# Autodesk Inventor assembly: ElectronicsHousing
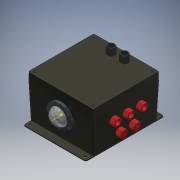
[picture p0: Inventor's stored thumbnail of the model, 180x180]
Saved by Autodesk Inventor 2018 (Build 220112000, 112)
## iProperties
Created: 2019-02-20
Part Number: ElectronicsHousing
Document SubType Name: Assembly
Designer: anirudh
Author: anirudh
## Documents named in this file (10)
- C:\Users\anirudh\Documents\MARS Fund\MATE Robotics\Silicon Sharks\2018-2019\ElectronicsHousing\ElectronicsHousing.iam
- C:\Users\anirudh\Documents\MARS Fund\MATE Robotics\Silicon Sharks\2018-2019\ElectronicsHousing\AluminumHousing(Master).ipt
- C:\Users\anirudh\Documents\MARS Fund\MATE Robotics\Silicon Sharks\2018-2019\ElectronicsHousing\Dome(2in)\2inDome.iam
- C:\Users\anirudh\Documents\MARS Fund\MATE Robotics\Silicon Sharks\2018-2019\ElectronicsHousing\Dome(2in)\DomeGasket.ipt
- C:\Users\anirudh\Documents\MARS Fund\MATE Robotics\Silicon Sharks\2018-2019\ElectronicsHousing\PENETRATOR-M-BOLT-6MM-10-25-R2.ipt
- C:\Users\anirudh\Documents\MARS Fund\MATE Robotics\Silicon Sharks\2018-2019\ElectronicsHousing\6mmPenetratorORing.ipt
- C:\Users\anirudh\Documents\MARS Fund\MATE Robotics\Silicon Sharks\2018-2019\ElectronicsHousing\PENETRATOR-M-BOLT-8MM-10-25-R1.ipt
- C:\Users\anirudh\Documents\MARS Fund\MATE Robotics\Silicon Sharks\2018-2019\ElectronicsHousing\CELSIUS-TEMPERATURE-SENSOR-ASSEMBLY-X1.ipt
- C:\Users\anirudh\Documents\MARS Fund\MATE Robotics\Silicon Sharks\2018-2019\ElectronicsHousing\BAR30-SENSOR-ASSEMBLY-R1.ipt
- C:\Users\anirudh\Documents\MARS Fund\MATE Robotics\Silicon Sharks\2018-2019\ElectronicsHousing\PENETRATOR-M-BLANK-10-25-R3.ipt
## Components (30 placed, 9 different names)
1. AluminumHousing(Master):1 — Mate:11, Mate:12, Mate:16, Mate:17, Mate:18, Mate:19, Mate:20, Mate:36, Mate:37, Mate:38, Mate:45, Mate:47, Mate:49, Mate:53, Mate:54, Mate:55, Mate:56, Mate:57, Mate:58, Mate:59, Mate:60, Mate:63, Mate:64, Mate:70, Mate:71, Mate:72, Mate:73, Mate:76, Mate:77, Mate:80, Mate:81
2. 2inDome:1 [sub-assembly] — Mate:1, Mate:2, Mate:3, Mate:4, Mate:5, Mate:12, Mate:13, Mate:14, Mate:15, Mate:16, Mate:17, Mate:18
3. DomeGasket:1 — Mate:1, Mate:2, Mate:3, Mate:4, Mate:5, Mate:11, Mate:13, Mate:14, Mate:15
4. 2inDome:2 [sub-assembly] — Mate:6, Mate:7, Mate:8, Mate:9, Mate:10, Mate:20, Mate:21, Mate:22, Mate:23
5. DomeGasket:2 — Mate:6, Mate:7, Mate:8, Mate:9, Mate:10, Mate:19, Mate:21, Mate:22, Mate:23
6. PENETRATOR-M-BOLT-6MM-10-25-R2:1 — Flush:2, Mate:30, Mate:31, Mate:36, Mate:56
7. PENETRATOR-M-BOLT-6MM-10-25-R2:2 — Flush:1, Flush:2, Mate:32, Mate:33, Mate:37, Mate:55
8. PENETRATOR-M-BOLT-6MM-10-25-R2:3 — Flush:1, Mate:34, Mate:35, Mate:38, Mate:54
9. 6mmPenetratorORing:1 — Mate:30, Mate:31
10. 6mmPenetratorORing:2 — Mate:32, Mate:33
11. 6mmPenetratorORing:3 — Mate:34, Mate:35
12. 6mmPenetratorORing:4 — Mate:39, Mate:40
13. PENETRATOR-M-BOLT-6MM-10-25-R2:4 — Mate:39, Mate:40, Mate:45, Flush:3, Mate:59
14. 6mmPenetratorORing:5 — Mate:41, Mate:42
15. PENETRATOR-M-BOLT-6MM-10-25-R2:5 — Mate:41, Mate:42, Mate:47, Flush:3, Flush:4, Mate:58
16. 6mmPenetratorORing:6 — Mate:43, Mate:44
17. PENETRATOR-M-BOLT-6MM-10-25-R2:6 — Mate:43, Mate:44, Mate:49, Flush:4, Mate:57
18. PENETRATOR-M-BOLT-8MM-10-25-R1:1 — Mate:51, Mate:52, Mate:53, Mate:60, Flush:5
19. 6mmPenetratorORing:7 — Mate:51, Mate:52
20. 6mmPenetratorORing:8 — Mate:61, Mate:62
21. PENETRATOR-M-BOLT-8MM-10-25-R1:2 — Mate:61, Mate:62, Mate:63, Mate:64, Flush:5
22. CELSIUS-TEMPERATURE-SENSOR-ASSEMBLY-X1:1 — Flush:6, Mate:69, Mate:73, Flush:8
23. BAR30-SENSOR-ASSEMBLY-R1:1 — Mate:65, Mate:66, Mate:70, Mate:71, Flush:7
24. 6mmPenetratorORing:9 — Mate:67, Mate:68
25. PENETRATOR-M-BOLT-6MM-10-25-R2:7 — Mate:67, Mate:68, Flush:6, Mate:69, Mate:72
26. 6mmPenetratorORing:10 — Mate:65, Mate:66
27. PENETRATOR-M-BLANK-10-25-R3:1 — Mate:74, Mate:75, Mate:76, Mate:77, Flush:7
28. PENETRATOR-M-BLANK-10-25-R3:2 — Mate:78, Mate:79, Mate:80, Mate:81, Flush:8
29. 6mmPenetratorORing:11 — Mate:74, Mate:75
30. 6mmPenetratorORing:12 — Mate:78, Mate:79
## Relationships (80: Mate 72, Flush 8)
- Mate:1: 2inDome:1 ↔ DomeGasket:1
- Mate:2: 2inDome:1 ↔ DomeGasket:1
- Mate:3: 2inDome:1 ↔ DomeGasket:1
- Mate:4: 2inDome:1 ↔ DomeGasket:1
- Mate:5: 2inDome:1 ↔ DomeGasket:1
- Mate:6: 2inDome:2 ↔ DomeGasket:2
- Mate:7: 2inDome:2 ↔ DomeGasket:2
- Mate:8: 2inDome:2 ↔ DomeGasket:2
- Mate:9: 2inDome:2 ↔ DomeGasket:2
- Mate:10: 2inDome:2 ↔ DomeGasket:2
- Mate:11: AluminumHousing(Master):1 ↔ DomeGasket:1
- Mate:12: AluminumHousing(Master):1 ↔ 2inDome:1
- Mate:13: 2inDome:1 ↔ DomeGasket:1
- Mate:14: 2inDome:1 ↔ DomeGasket:1
- Mate:15: 2inDome:1 ↔ DomeGasket:1
- Mate:16: AluminumHousing(Master):1 ↔ 2inDome:1
- Mate:17: AluminumHousing(Master):1 ↔ 2inDome:1
- Mate:18: AluminumHousing(Master):1 ↔ 2inDome:1
- Mate:19: AluminumHousing(Master):1 ↔ DomeGasket:2
- Mate:20: AluminumHousing(Master):1 ↔ 2inDome:2
- Mate:21: 2inDome:2 ↔ DomeGasket:2
- Mate:22: 2inDome:2 ↔ DomeGasket:2
- Mate:23: 2inDome:2 ↔ DomeGasket:2
- Flush:1: PENETRATOR-M-BOLT-6MM-10-25-R2:2 ↔ PENETRATOR-M-BOLT-6MM-10-25-R2:3
- Flush:2: PENETRATOR-M-BOLT-6MM-10-25-R2:1 ↔ PENETRATOR-M-BOLT-6MM-10-25-R2:2
- Mate:30: PENETRATOR-M-BOLT-6MM-10-25-R2:1 ↔ 6mmPenetratorORing:1
- Mate:31: PENETRATOR-M-BOLT-6MM-10-25-R2:1 ↔ 6mmPenetratorORing:1
- Mate:32: PENETRATOR-M-BOLT-6MM-10-25-R2:2 ↔ 6mmPenetratorORing:2
- Mate:33: PENETRATOR-M-BOLT-6MM-10-25-R2:2 ↔ 6mmPenetratorORing:2
- Mate:34: PENETRATOR-M-BOLT-6MM-10-25-R2:3 ↔ 6mmPenetratorORing:3
- Mate:35: PENETRATOR-M-BOLT-6MM-10-25-R2:3 ↔ 6mmPenetratorORing:3
- Mate:36: AluminumHousing(Master):1 ↔ PENETRATOR-M-BOLT-6MM-10-25-R2:1
- Mate:37: AluminumHousing(Master):1 ↔ PENETRATOR-M-BOLT-6MM-10-25-R2:2
- Mate:38: AluminumHousing(Master):1 ↔ PENETRATOR-M-BOLT-6MM-10-25-R2:3
- Mate:39: 6mmPenetratorORing:4 ↔ PENETRATOR-M-BOLT-6MM-10-25-R2:4
- Mate:40: 6mmPenetratorORing:4 ↔ PENETRATOR-M-BOLT-6MM-10-25-R2:4
- Mate:41: 6mmPenetratorORing:5 ↔ PENETRATOR-M-BOLT-6MM-10-25-R2:5
- Mate:42: 6mmPenetratorORing:5 ↔ PENETRATOR-M-BOLT-6MM-10-25-R2:5
- Mate:43: 6mmPenetratorORing:6 ↔ PENETRATOR-M-BOLT-6MM-10-25-R2:6
- Mate:44: 6mmPenetratorORing:6 ↔ PENETRATOR-M-BOLT-6MM-10-25-R2:6
- Mate:45: AluminumHousing(Master):1 ↔ PENETRATOR-M-BOLT-6MM-10-25-R2:4
- Mate:47: AluminumHousing(Master):1 ↔ PENETRATOR-M-BOLT-6MM-10-25-R2:5
- Flush:3: PENETRATOR-M-BOLT-6MM-10-25-R2:4 ↔ PENETRATOR-M-BOLT-6MM-10-25-R2:5
- Mate:49: AluminumHousing(Master):1 ↔ PENETRATOR-M-BOLT-6MM-10-25-R2:6
- Flush:4: PENETRATOR-M-BOLT-6MM-10-25-R2:5 ↔ PENETRATOR-M-BOLT-6MM-10-25-R2:6
- Mate:51: PENETRATOR-M-BOLT-8MM-10-25-R1:1 ↔ 6mmPenetratorORing:7
- Mate:52: PENETRATOR-M-BOLT-8MM-10-25-R1:1 ↔ 6mmPenetratorORing:7
- Mate:53: AluminumHousing(Master):1 ↔ PENETRATOR-M-BOLT-8MM-10-25-R1:1
- Mate:54: AluminumHousing(Master):1 ↔ PENETRATOR-M-BOLT-6MM-10-25-R2:3
- Mate:55: AluminumHousing(Master):1 ↔ PENETRATOR-M-BOLT-6MM-10-25-R2:2
- Mate:56: AluminumHousing(Master):1 ↔ PENETRATOR-M-BOLT-6MM-10-25-R2:1
- Mate:57: AluminumHousing(Master):1 ↔ PENETRATOR-M-BOLT-6MM-10-25-R2:6
- Mate:58: AluminumHousing(Master):1 ↔ PENETRATOR-M-BOLT-6MM-10-25-R2:5
- Mate:59: AluminumHousing(Master):1 ↔ PENETRATOR-M-BOLT-6MM-10-25-R2:4
- Mate:60: AluminumHousing(Master):1 ↔ PENETRATOR-M-BOLT-8MM-10-25-R1:1
- Mate:61: 6mmPenetratorORing:8 ↔ PENETRATOR-M-BOLT-8MM-10-25-R1:2
- Mate:62: 6mmPenetratorORing:8 ↔ PENETRATOR-M-BOLT-8MM-10-25-R1:2
- Mate:63: AluminumHousing(Master):1 ↔ PENETRATOR-M-BOLT-8MM-10-25-R1:2
- Mate:64: AluminumHousing(Master):1 ↔ PENETRATOR-M-BOLT-8MM-10-25-R1:2
- Flush:5: PENETRATOR-M-BOLT-8MM-10-25-R1:1 ↔ PENETRATOR-M-BOLT-8MM-10-25-R1:2
- Mate:65: BAR30-SENSOR-ASSEMBLY-R1:1 ↔ 6mmPenetratorORing:10
- Mate:66: BAR30-SENSOR-ASSEMBLY-R1:1 ↔ 6mmPenetratorORing:10
- Mate:67: 6mmPenetratorORing:9 ↔ PENETRATOR-M-BOLT-6MM-10-25-R2:7
- Mate:68: 6mmPenetratorORing:9 ↔ PENETRATOR-M-BOLT-6MM-10-25-R2:7
- Flush:6: CELSIUS-TEMPERATURE-SENSOR-ASSEMBLY-X1:1 ↔ PENETRATOR-M-BOLT-6MM-10-25-R2:7
- Mate:69: CELSIUS-TEMPERATURE-SENSOR-ASSEMBLY-X1:1 ↔ PENETRATOR-M-BOLT-6MM-10-25-R2:7
- Mate:70: AluminumHousing(Master):1 ↔ BAR30-SENSOR-ASSEMBLY-R1:1
- Mate:71: AluminumHousing(Master):1 ↔ BAR30-SENSOR-ASSEMBLY-R1:1
- Mate:72: AluminumHousing(Master):1 ↔ PENETRATOR-M-BOLT-6MM-10-25-R2:7
- Mate:73: AluminumHousing(Master):1 ↔ CELSIUS-TEMPERATURE-SENSOR-ASSEMBLY-X1:1
- Mate:74: PENETRATOR-M-BLANK-10-25-R3:1 ↔ 6mmPenetratorORing:11
- Mate:75: PENETRATOR-M-BLANK-10-25-R3:1 ↔ 6mmPenetratorORing:11
- Mate:76: AluminumHousing(Master):1 ↔ PENETRATOR-M-BLANK-10-25-R3:1
- Mate:77: AluminumHousing(Master):1 ↔ PENETRATOR-M-BLANK-10-25-R3:1
- Flush:7: BAR30-SENSOR-ASSEMBLY-R1:1 ↔ PENETRATOR-M-BLANK-10-25-R3:1
- Mate:78: PENETRATOR-M-BLANK-10-25-R3:2 ↔ 6mmPenetratorORing:12
- Mate:79: PENETRATOR-M-BLANK-10-25-R3:2 ↔ 6mmPenetratorORing:12
- Mate:80: AluminumHousing(Master):1 ↔ PENETRATOR-M-BLANK-10-25-R3:2
- Mate:81: AluminumHousing(Master):1 ↔ PENETRATOR-M-BLANK-10-25-R3:2
- Flush:8: CELSIUS-TEMPERATURE-SENSOR-ASSEMBLY-X1:1 ↔ PENETRATOR-M-BLANK-10-25-R3:2
